# Autodesk Inventor assembly: Rover_construction_2.0
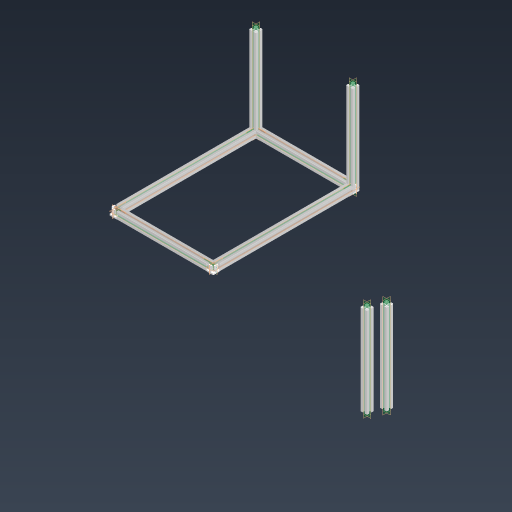
[picture p0: Inventor's stored thumbnail of the model, 512x512]
Saved by Autodesk Inventor 2023.2 (Build 272271030, 271C)
## iProperties
Created: 2025-08-18
Part Number: Rover_construction_2.0
Document SubType Name: Assembly
Designer: Олег Коноваленко
Author: Олег Коноваленко
## Documents named in this file (4)
- D:\!Rover\Rover\Rover_construction\Rover_construction_2.0.iam
- Rover_2.0.iam
- C:\Users\I9232\Downloads\3-х сторонний соединитель 30х30\3-х сторонний соединитель 30х30.ipt
- D:\!Rover\Rover\Rover_construction\Профиль 30x30\Профиль 30x30.ipt
## Components (12 placed, 2 different names)
1. 3-х сторонний соединитель 30х30:1 — Заподлицо:4, Заподлицо:5, Совмещение:4, Заподлицо:6, Заподлицо:7, Совмещение:5, Совмещение:12, Заподлицо:11, Совмещение:13
2. 3-х сторонний соединитель 30х30:2 — Заподлицо:8, Совмещение:6, Совмещение:7, Совмещение:8, Заподлицо:9, Совмещение:9
3. 3-х сторонний соединитель 30х30:3 — Совмещение:1, Заподлицо:1, Совмещение:2, Заподлицо:2, Заподлицо:3, Совмещение:3, Заподлицо:12, Заподлицо:13, Совмещение:14
4. 3-х сторонний соединитель 30х30:4 — Заподлицо:10, Совмещение:10, Совмещение:11
5. Профиль 30x30:1 — Заподлицо:6, Заподлицо:7, Совмещение:5, Совмещение:10, Совмещение:11
6. Профиль 30x30:2 — Заподлицо:2, Заподлицо:3, Совмещение:3, Заподлицо:8, Совмещение:6, Совмещение:7
7. Профиль 30x30:3 — Совмещение:1, Заподлицо:1, Совмещение:2, Заподлицо:4, Заподлицо:5, Совмещение:4
8. Профиль 30x30:4 — Совмещение:8, Заподлицо:9, Совмещение:9, Заподлицо:10
9. Профиль 30x30:5 — Заподлицо:12, Заподлицо:13, Совмещение:14
10. Профиль 30x30:6
11. Профиль 30x30:7
12. Профиль 30x30:8 — Совмещение:12, Заподлицо:11, Совмещение:13
## Relationships (27: Mate 14, Flush 13)
- Совмещение:1 [Mate]: 3-х сторонний соединитель 30х30:3 ↔ Профиль 30x30:3
- Заподлицо:1 [Flush]: 3-х сторонний соединитель 30х30:3 ↔ Профиль 30x30:3
- Совмещение:2 [Mate]: 3-х сторонний соединитель 30х30:3 ↔ Профиль 30x30:3
- Заподлицо:2 [Flush]: 3-х сторонний соединитель 30х30:3 ↔ Профиль 30x30:2
- Заподлицо:3 [Flush]: 3-х сторонний соединитель 30х30:3 ↔ Профиль 30x30:2
- Совмещение:3 [Mate]: 3-х сторонний соединитель 30х30:3 ↔ Профиль 30x30:2
- Заподлицо:4 [Flush]: 3-х сторонний соединитель 30х30:1 ↔ Профиль 30x30:3
- Заподлицо:5 [Flush]: 3-х сторонний соединитель 30х30:1 ↔ Профиль 30x30:3
- Совмещение:4 [Mate]: 3-х сторонний соединитель 30х30:1 ↔ Профиль 30x30:3
- Заподлицо:6 [Flush]: 3-х сторонний соединитель 30х30:1 ↔ Профиль 30x30:1
- Заподлицо:7 [Flush]: 3-х сторонний соединитель 30х30:1 ↔ Профиль 30x30:1
- Совмещение:5 [Mate]: 3-х сторонний соединитель 30х30:1 ↔ Профиль 30x30:1
- Заподлицо:8 [Flush]: 3-х сторонний соединитель 30х30:2 ↔ Профиль 30x30:2
- Совмещение:6 [Mate]: 3-х сторонний соединитель 30х30:2 ↔ Профиль 30x30:2
- Совмещение:7 [Mate]: 3-х сторонний соединитель 30х30:2 ↔ Профиль 30x30:2
- Совмещение:8 [Mate]: 3-х сторонний соединитель 30х30:2 ↔ Профиль 30x30:4
- Заподлицо:9 [Flush]: 3-х сторонний соединитель 30х30:2 ↔ Профиль 30x30:4
- Совмещение:9 [Mate]: 3-х сторонний соединитель 30х30:2 ↔ Профиль 30x30:4
- Заподлицо:10 [Flush]: 3-х сторонний соединитель 30х30:4 ↔ Профиль 30x30:4
- Совмещение:10 [Mate]: 3-х сторонний соединитель 30х30:4 ↔ Профиль 30x30:1
- Совмещение:11 [Mate]: 3-х сторонний соединитель 30х30:4 ↔ Профиль 30x30:1
- Совмещение:12 [Mate]: 3-х сторонний соединитель 30х30:1 ↔ Профиль 30x30:8
- Заподлицо:11 [Flush]: 3-х сторонний соединитель 30х30:1 ↔ Профиль 30x30:8
- Совмещение:13 [Mate]: 3-х сторонний соединитель 30х30:1 ↔ Профиль 30x30:8
- Заподлицо:12 [Flush]: 3-х сторонний соединитель 30х30:3 ↔ Профиль 30x30:5
- Заподлицо:13 [Flush]: 3-х сторонний соединитель 30х30:3 ↔ Профиль 30x30:5
- Совмещение:14 [Mate]: 3-х сторонний соединитель 30х30:3 ↔ Профиль 30x30:5
